# Autodesk Inventor assembly: Egg Capsule
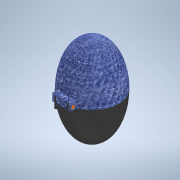
[picture p0: Inventor's stored thumbnail of the model, 180x180]
Saved by Autodesk Inventor 2022 (Build 260153000, 153)
## iProperties
Created: 2022-02-15
Part Number: Egg Capsule
Document SubType Name: Assembly
Designer: Nathan Griffith
Author: Nathan Griffith
## Documents named in this file (4)
- C:\Users\Nathan Griffith\Documents\Inventor\Physics Egg Drop\Egg Capsule.iam
- C:\Users\Nathan Griffith\Documents\Inventor\Physics Egg Drop\Egg capsule bottom.ipt
- C:\Users\Nathan Griffith\Documents\Inventor\Physics Egg Drop\Egg Capsule Top.ipt
- C:\Users\Nathan Griffith\Documents\Inventor\Physics Egg Drop\Nuts n Bolts n Stuff\Pin .5 in by .1 in.ipt
## Components (3 placed, 3 different names)
1. Egg capsule bottom:1 — Insert:2
2. Egg Capsule Top:1 — Insert:1, Insert:2
3. Pin .5 in by .1 in:1 — Insert:1
## Relationships (2: Insert 2)
- Insert:1: Egg Capsule Top:1 ↔ Pin .5 in by .1 in:1
- Insert:2: Egg capsule bottom:1 ↔ Egg Capsule Top:1
